# Autodesk Inventor assembly: 初段_多段ギア
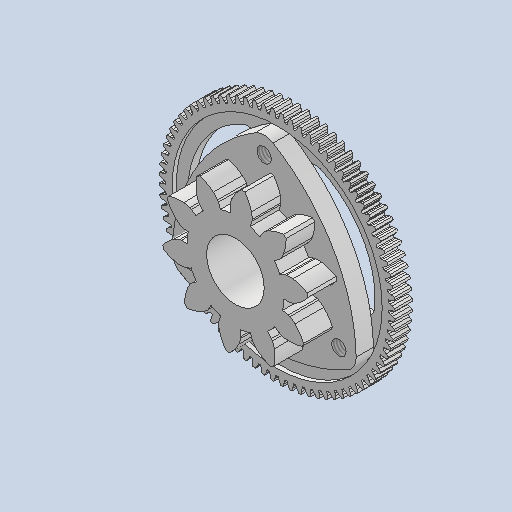
[picture p0: Inventor's stored thumbnail of the model, 512x512]
Saved by Autodesk Inventor 2022.2 (Build 262287000, 287)
## iProperties
Created: 2022-01-11
Part Number: 初段_多段ギア
Document SubType Name: Assembly
Designer: acps
Author: acps
## Documents named in this file (3)
- C:\Users\acps\Documents\srdc\srdc_ksh\ギア\初段_多段ギア.iam
- C:\Users\acps\Documents\srdc\srdc_ksh\ギア\多段ギアm2z10t8.ipt
- C:\Users\acps\Documents\srdc\srdc_ksh\ギア\初段ギアm0.5z80.ipt
## Components (2 placed, 2 different names)
1. 多段ギアm2z10t8:1 — Mate:1, Mate:2, Insert:1
2. 初段ギアm0.5z80:1 — Mate:1, Mate:2, Insert:1
## Relationships (3: Mate 2, Insert 1)
- Mate:1: 多段ギアm2z10t8:1 ↔ 初段ギアm0.5z80:1
- Mate:2: 多段ギアm2z10t8:1 ↔ 初段ギアm0.5z80:1
- Insert:1: 多段ギアm2z10t8:1 ↔ 初段ギアm0.5z80:1
